# Autodesk Inventor assembly: prototipo
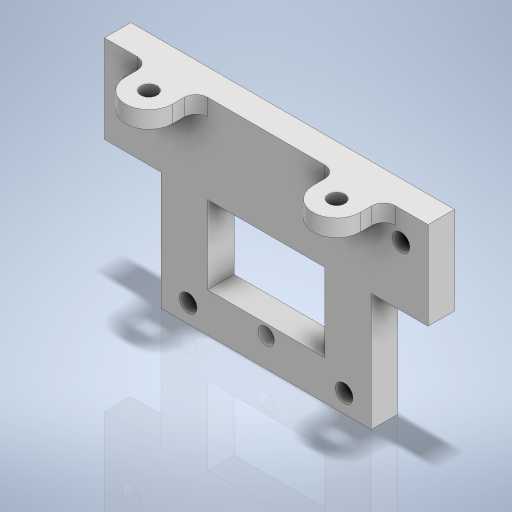
[picture p0: Inventor's stored thumbnail of the model, 512x512]
Saved by Autodesk Inventor 2024.3 (Build 283343000, 343)
## iProperties
Created: 2024-03-02
Part Number: prototipo
Document SubType Name: Assembly
Designer: joaov
Author: joaov
## Documents named in this file (6)
- D:\Downloads\IC\Bancada\protoripo\prototipo.iam
- D:\Downloads\IC\Bancada\protoripo\corpo.ipt
- D:\Downloads\IC\Bancada\protoripo\tampa.ipt
- D:\Downloads\IC\Bancada\protoripo\tampa_2.ipt
- D:\Downloads\IC\Bancada\protoripo\bloco_aquecimento.ipt
- D:\Downloads\IC\Bancada\protoripo\ventilador.ipt
## Components (5 placed, 5 different names)
1. corpo:1 — Coincidente:2, Coincidente:3, Coincidente:4, Coincidente:5
2. tampa_1 — Coincidente:2, Coincidente:3
3. tampa_2 — Coincidente:4, Coincidente:5, Coincidente:8, Coincidente:10, Coincidente:11
4. bloco_aquecimento:1 — Coincidente:10, Coincidente:11
5. ventilador:1 — Coincidente:8
## Relationships (7: Mate 7)
- Coincidente:2 [Mate]: corpo:1 ↔ tampa_1
- Coincidente:3 [Mate]: corpo:1 ↔ tampa_1
- Coincidente:4 [Mate]: corpo:1 ↔ tampa_2
- Coincidente:5 [Mate]: corpo:1 ↔ tampa_2
- Coincidente:8 [Mate]: tampa_2 ↔ ventilador:1
- Coincidente:10 [Mate]: tampa_2 ↔ bloco_aquecimento:1
- Coincidente:11 [Mate]: tampa_2 ↔ bloco_aquecimento:1
